# Autodesk Inventor assembly: Antrieb final
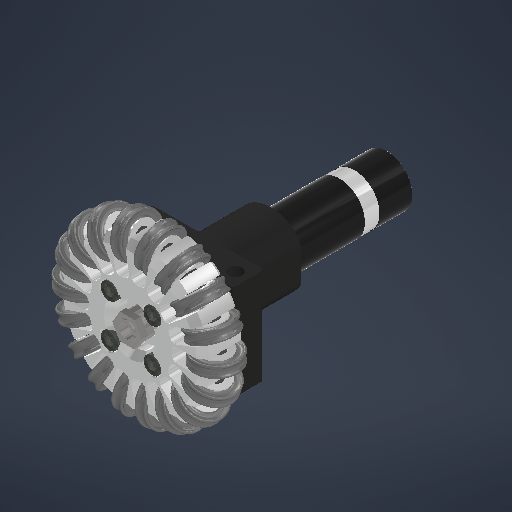
[picture p0: Inventor's stored thumbnail of the model, 512x512]
Saved by Autodesk Inventor 2025.3 (Build 293356000, 356)
## iProperties
Created: 2025-03-03
Part Number: Antrieb final
Document SubType Name: Assembly
Designer: theod
Author: theod
## Documents named in this file (4)
- C:\Users\theod\Desktop\Team Mathimazierer v2025\Antrieb final.iam
- C:\Users\theod\Desktop\Team Mathimazierer v2025\gute motorhalterung von faaaaabs.ipt
- C:\Users\theod\Desktop\Team Mathimazierer v2025\Maxon EC-16 30W(1).iam
- C:\Users\theod\Desktop\Team Mathimazierer v2025\RadLWL.iam
## Components (3 placed, 3 different names)
1. gute motorhalterung von faaaaabs:1 — Passend:1, Fluchtend:1, Passend:2, Passend:3, Passend:4, Passend:5, Passend:7, Winkel:1
2. Maxon EC-16 30W(1):1 [sub-assembly] — Passend:3, Passend:4, Passend:5, Passend:6
3. RadLWL:1 [sub-assembly] — Passend:6, Passend:7, Winkel:1
## Relationships (9: Mate 7, Flush 1, Angle 1)
- Passend:1 [Mate]: gute motorhalterung von faaaaabs:1
- Fluchtend:1 [Flush]: gute motorhalterung von faaaaabs:1
- Passend:2 [Mate]: gute motorhalterung von faaaaabs:1
- Passend:3 [Mate]: gute motorhalterung von faaaaabs:1 ↔ Maxon EC-16 30W(1):1
- Passend:4 [Mate]: gute motorhalterung von faaaaabs:1 ↔ Maxon EC-16 30W(1):1
- Passend:5 [Mate]: gute motorhalterung von faaaaabs:1 ↔ Maxon EC-16 30W(1):1
- Passend:6 [Mate]: Maxon EC-16 30W(1):1 ↔ RadLWL:1
- Passend:7 [Mate] (1 mm): gute motorhalterung von faaaaabs:1 ↔ RadLWL:1
- Winkel:1 [Angle] (90 deg): gute motorhalterung von faaaaabs:1 ↔ RadLWL:1
